# Autodesk Inventor assembly: Disc B Assembly
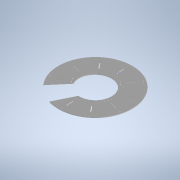
[picture p0: Inventor's stored thumbnail of the model, 180x180]
Saved by Autodesk Inventor 2020 (Build 240168000, 168)
## iProperties
Created: 2020-05-11
Part Number: Disc B Assembly
Document SubType Name: Assembly
Designer: Dan Wikman
Author: Dan Wikman
## Documents named in this file (5)
- C:\Users\Dan Wikman\OneDrive\University Life\2020, Semester 1\METR4900 Honours Thesis\Full Scale Design\Disc B Assembly.iam
- C:\Users\Dan Wikman\OneDrive\University Life\2020, Semester 1\METR4900 Honours Thesis\Full Scale Design\Platform B1.ipt
- C:\Users\Dan Wikman\OneDrive\University Life\2020, Semester 1\METR4900 Honours Thesis\Full Scale Design\Platform B2.ipt
- C:\Users\Dan Wikman\OneDrive\University Life\2020, Semester 1\METR4900 Honours Thesis\Full Scale Design\Platform B3.ipt
- C:\Users\Dan Wikman\OneDrive\University Life\2020, Semester 1\METR4900 Honours Thesis\Full Scale Design\Platform B4.ipt
## Components (4 placed, 4 different names)
1. Platform B1:1 — Flush:2, Mate:3, Mate:4
2. Platform B2:1 — Flush:1, Mate:1, Mate:2, Flush:3, Mate:5, Mate:6
3. Platform B3:1 — Flush:1, Mate:1, Mate:2, Flush:2, Mate:3, Mate:4
4. Platform B4:1 — Flush:3, Mate:5, Mate:6
## Relationships (9: Mate 6, Flush 3)
- Flush:1: Platform B2:1 ↔ Platform B3:1
- Mate:1: Platform B2:1 ↔ Platform B3:1
- Mate:2: Platform B2:1 ↔ Platform B3:1
- Flush:2: Platform B1:1 ↔ Platform B3:1
- Mate:3: Platform B1:1 ↔ Platform B3:1
- Mate:4: Platform B1:1 ↔ Platform B3:1
- Flush:3: Platform B2:1 ↔ Platform B4:1
- Mate:5: Platform B2:1 ↔ Platform B4:1
- Mate:6: Platform B2:1 ↔ Platform B4:1
